# Autodesk Inventor assembly: сборка ладони
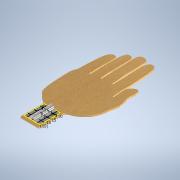
[picture p0: Inventor's stored thumbnail of the model, 180x180]
Saved by Autodesk Inventor 2020 (Build 240168000, 168)
## iProperties
Created: 2022-03-20
Part Number: сборка ладони
Document SubType Name: Assembly
Designer: Администратор
Author: Администратор
## Documents named in this file (3)
- \\sch239.net\UserHomes\Students\Other\glazovaes\сборка ладони.iam
- \\sch239.net\UserHomes\Students\Other\glazovaes\ладонь.ipt
- \\sch239.net\UserHomes\Students\Other\glazovaes\крепление направляющей руки.ipt
## Components (2 placed, 2 different names)
1. ладонь:1 — Совмещение:1, Совмещение:2
2. крепление направляющей руки:1 — Совмещение:1, Совмещение:2
## Relationships (2: Mate 2)
- Совмещение:1 [Mate]: ладонь:1 ↔ крепление направляющей руки:1
- Совмещение:2 [Mate]: ладонь:1 ↔ крепление направляющей руки:1
